# Autodesk Inventor assembly: pendulum
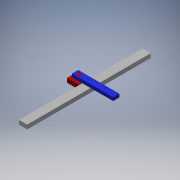
[picture p0: Inventor's stored thumbnail of the model, 180x180]
Saved by Autodesk Inventor 2017 (Build 210142000, 142)
## iProperties
Part Number: pendulum
Material: Generisch
Document SubType Name: Assembly
Designer: 10154704
Author: 10154704
## Documents named in this file (4)
- F:\LFuhrig\Master\InventorToSimscape\InversesPendel\invertedPendulum.iam
- F:\LFuhrig\Master\InventorToSimscape\InversesPendel\cart.ipt
- F:\LFuhrig\Master\InventorToSimscape\InversesPendel\pendulum.ipt
- F:\LFuhrig\Master\InventorToSimscape\InversesPendel\base.ipt
## Components (3 placed, 3 different names)
1. cart:1 — Fluchtend:2, Einfügen:1, Passend:3
2. pendulum:1 — Einfügen:1
3. base:1 — Passend:1, Passend:2, Fluchtend:3, Passend:3
## Relationships (6: Mate 3, Flush 2, Insert 1)
- Fluchtend:2 [Flush]: cart:1
- Einfügen:1 [Insert]: cart:1 ↔ pendulum:1
- Passend:1 [Mate]: base:1
- Passend:2 [Mate]: base:1
- Fluchtend:3 [Flush]: base:1
- Passend:3 [Mate]: cart:1 ↔ base:1
